# Autodesk Inventor assembly: CableBraider
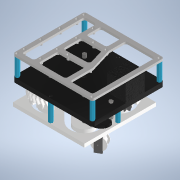
[picture p0: Inventor's stored thumbnail of the model, 180x180]
Saved by Autodesk Inventor 2021 (Build 250183000, 183)
## iProperties
Created: 2020-07-21
Part Number: CableBraider
Document SubType Name: Assembly
Designer: elmar
Author: elmar
## Documents named in this file (17)
- D:\FourWireBraidingMachine\InventorFiles\CableBraider.iam
- D:\FourWireBraidingMachine\InventorFiles\BasePlate.ipt
- D:\FourWireBraidingMachine\InventorFiles\DriveGear.ipt
- D:\FourWireBraidingMachine\InventorFiles\HornGear.ipt
- D:\FourWireBraidingMachine\InventorFiles\Standoff.ipt
- D:\FourWireBraidingMachine\InventorFiles\ReductionGearBracket.ipt
- D:\FourWireBraidingMachine\InventorFiles\ReductionGear.ipt
- D:\FourWireBraidingMachine\InventorFiles\ReductionDriveGear.ipt
- D:\FourWireBraidingMachine\InventorFiles\WinderAssembly.iam
- C:\Users\elmar\OneDrive\Documents\Inventor\Content Center Files\R2021\en-US\ANSI B18.2.4.2M\ANSI B18.2.4.2M - M8x1.25 - 13.ipt
- D:\FourWireBraidingMachine\InventorFiles\Carriage.iam
- C:\Users\elmar\OneDrive\Documents\Inventor\Content Center Files\R2021\en-US\AS 1237 (2.1)\AS 1237 - 8.ipt
- C:\Users\elmar\OneDrive\Documents\Inventor\Content Center Files\R2021\en-US\AS 1112 (2)\AS 1112 - M8  Type 5.ipt
- D:\FourWireBraidingMachine\InventorFiles\GuidePlateV0.ipt
- C:\Users\elmar\OneDrive\Documents\Inventor\Content Center Files\R2021\en-US\DIN 976-1 A\DIN 976-1 - M8 x 70 - A.ipt
- D:\FourWireBraidingMachine\InventorFiles\NEMA17.ipt
- D:\FourWireBraidingMachine\InventorFiles\ElectronicsPlate.ipt
## Components (39 placed, 16 different names)
1. BasePlate:1 — Mate:1, Mate:2, Mate:3, Insert:3, Insert:5, Angle:1, Insert:15, Insert:17, Insert:18, Insert:21, Insert:22, Insert:23, Insert:24, Insert:25, Insert:26, Insert:28, Insert:38, Flush:1, Flush:2, Mate:4, Mate:7, Insert:41, Angle:4
2. DriveGear:1 — Mate:7, Mate:8
3. HornGear:1 — Insert:3, Angle:3, Mate:8
4. Standoff:1 — Insert:5
5. GuidePlateV0:1 — Flush:1, Flush:2, Mate:4, Mate:5, Tangent:1, Tangent:2
6. ReductionGearBracket:1 — Angle:1, Insert:12, Insert:15, Insert:33
7. ReductionDriveGear:1 — Insert:12
8. ReductionGear:1 — Insert:33, Insert:36
9. Standoff:2 — Insert:17
10. HornGear:2 — Insert:18, Angle:3
11. Standoff:3 — Insert:21
12. Standoff:4 — Insert:23, Flush:3
13. Standoff:5 — Insert:25
14. Standoff:6 — Insert:22
15. Standoff:7 — Insert:24
16. Standoff:8 — Insert:26
17. WinderAssembly:1 [sub-assembly]
18. ANSI B18.2.4.2M M8x1.25:2 — Insert:35
19. AS 1237 (2.1) 8:1 — Insert:35
20. ANSI B18.2.4.2M M8x1.25:3 — Insert:36
21. DIN 976-1 A M8 x 70:1 — Insert:39
22. NEMA17:1 — Insert:41, Angle:4
23. ElectronicsPlate:1 — Flush:3
24. ANSI B18.2.4.2M M8x1.25:1 — Insert:28, Insert:39
25. ANSI B18.2.4.2M M8x1.25:4
26. DIN 976-1 A M8 x 70:3 — Insert:40
27. DIN 976-1 A M8 x 70:4
28. DIN 976-1 A M8 x 70:5
29. DIN 976-1 A M8 x 70:6
30. Carriage:1 [sub-assembly] — Mate:5, Tangent:1, Tangent:2, Mate:6
31. Carriage:8 [sub-assembly]
32. AS 1112 (2) - Metric M8  Type 5:1 — Insert:38
33. AS 1112 (2) - Metric M8  Type 5:2
34. AS 1112 (2) - Metric M8  Type 5:3 — Insert:40
35. AS 1112 (2) - Metric M8  Type 5:4
36. AS 1112 (2) - Metric M8  Type 5:5
37. AS 1112 (2) - Metric M8  Type 5:6
38. AS 1112 (2) - Metric M8  Type 5:7
39. AS 1112 (2) - Metric M8  Type 5:8
## Component patterns: (2 elements, first: ANSI B18.2.4.2M M8x1.25:1), (4 elements, first: DIN 976-1 A M8 x 70:3), (2 elements, first: Carriage:1), (4 elements, first: AS 1112 (2) - Metric M8  Type 5:1), Component Pattern 1:2 (4 elements)
## Relationships (36: Insert 20, Mate 8, Angle 3, Flush 3, Tangent 2)
- Mate:1: BasePlate:1
- Mate:2: BasePlate:1
- Mate:3: BasePlate:1
- Insert:3 (1 mm): BasePlate:1 ↔ HornGear:1
- Insert:5: BasePlate:1 ↔ Standoff:1
- Angle:1 (0 deg): BasePlate:1 ↔ ReductionGearBracket:1
- Insert:12 (1 mm): ReductionGearBracket:1 ↔ ReductionDriveGear:1
- Insert:15: BasePlate:1 ↔ ReductionGearBracket:1
- Insert:17: BasePlate:1 ↔ Standoff:2
- Insert:18 (1 mm): BasePlate:1 ↔ HornGear:2
- Insert:21: BasePlate:1 ↔ Standoff:3
- Insert:22: BasePlate:1 ↔ Standoff:6
- Insert:23: BasePlate:1 ↔ Standoff:4
- Insert:24: BasePlate:1 ↔ Standoff:7
- Insert:25: BasePlate:1 ↔ Standoff:5
- Insert:26: BasePlate:1 ↔ Standoff:8
- Insert:28: BasePlate:1 ↔ ANSI B18.2.4.2M M8x1.25:1
- Insert:33 (1 mm): ReductionGearBracket:1 ↔ ReductionGear:1
- Insert:35: ANSI B18.2.4.2M M8x1.25:2 ↔ AS 1237 (2.1) 8:1
- Insert:36: ReductionGear:1 ↔ ANSI B18.2.4.2M M8x1.25:3
- Insert:38: BasePlate:1 ↔ AS 1112 (2) - Metric M8  Type 5:1
- Insert:39: DIN 976-1 A M8 x 70:1 ↔ ANSI B18.2.4.2M M8x1.25:1
- Insert:40: DIN 976-1 A M8 x 70:3 ↔ AS 1112 (2) - Metric M8  Type 5:3
- Flush:1: BasePlate:1 ↔ GuidePlateV0:1
- Flush:2: BasePlate:1 ↔ GuidePlateV0:1
- Mate:4 (40 mm): BasePlate:1 ↔ GuidePlateV0:1
- Mate:5: GuidePlateV0:1 ↔ Carriage:1
- Tangent:1: GuidePlateV0:1 ↔ Carriage:1
- Tangent:2: GuidePlateV0:1 ↔ Carriage:1
- Mate:6: Carriage:1
- Angle:3 (0 deg): HornGear:1 ↔ HornGear:2
- Mate:7: BasePlate:1 ↔ DriveGear:1
- Mate:8: DriveGear:1 ↔ HornGear:1
- Insert:41: BasePlate:1 ↔ NEMA17:1
- Angle:4 (0 deg): BasePlate:1 ↔ NEMA17:1
- Flush:3: Standoff:4 ↔ ElectronicsPlate:1
